# Autodesk Inventor assembly: Assembly4
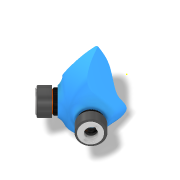
[picture p0: Inventor's stored thumbnail of the model, 180x180]
Saved by Autodesk Inventor 2021 (Build 250183000, 183)
## iProperties
Created: 2020-07-12
Part Number: Assembly4
Document SubType Name: Assembly
Designer: Derm
Author: Derm
## Documents named in this file (10)
- C:\Users\Derm\n95\v7\Assembly4.iam
- C:\Users\Derm\n95\v7\maskBodyV4Molds\thermoformedSupport.ipt
- C:\Users\Derm\n95\v7\3dpBayonetteMountV1Fastener.ipt
- C:\Users\Derm\n95\v7\3dpBayonetteMountV2.ipt
- C:\Users\Derm\n95\v7\outerMountGasket.ipt
- C:\Users\Derm\n95\v7\maskBodyV4Molds\main.ipt
- C:\Users\Derm\n95\v7\cartMount.ipt
- C:\Users\Derm\n95\v7\cartCap.ipt
- C:\Users\Derm\n95\v7\1inFilterInsert.ipt
- C:\Users\Derm\n95\v7\1inFilterInsertGasket.ipt
## Components (15 placed, 9 different names)
1. thermoformedSupport:1 — Mate:3, Mate:6, Mate:7, Mate:8, Mate:11, Mate:12, Flush:1, Flush:2
2. 3dpBayonetteMountV1Fastener:1 — Mate:5, Mate:7, Mate:10, Mate:18
3. 3dpBayonetteMountV2:1 — Mate:4, Mate:5, Mate:6, Mate:11, Mate:13, Mate:14, Mate:15
4. outerMountGasket:1 — Mate:4, Mate:10, Mate:17
5. 3dpBayonetteMountV1Fastener:2 — Mate:2, Mate:8, Mate:9, Mate:19
6. 3dpBayonetteMountV2:2 — Mate:1, Mate:3, Mate:12, Mate:16
7. outerMountGasket:2 — Mate:1, Mate:2, Mate:9
8. main:1 — Flush:1, Flush:2, Mate:14, Mate:15, Mate:16, Mate:18
9. cartMount:1 — Mate:13, Mate:17, Mate:21, Mate:22, Mate:25
10. cartMount:2 — Mate:19, Mate:20
11. cartCap:1 — Mate:21
12. cartCap:2 — Mate:20
13. 1inFilterInsert:1 — Mate:22, Flush:3, Mate:23
14. 1inFilterInsertGasket:1 — Flush:3, Mate:24, Mate:25
15. 1inFilterInsertGasket:2 — Mate:23, Mate:24
## Relationships (28: Mate 25, Flush 3)
- Mate:1: 3dpBayonetteMountV2:2 ↔ outerMountGasket:2
- Mate:2: 3dpBayonetteMountV1Fastener:2 ↔ outerMountGasket:2
- Mate:3: thermoformedSupport:1 ↔ 3dpBayonetteMountV2:2
- Mate:4: 3dpBayonetteMountV2:1 ↔ outerMountGasket:1
- Mate:5: 3dpBayonetteMountV1Fastener:1 ↔ 3dpBayonetteMountV2:1
- Mate:6: thermoformedSupport:1 ↔ 3dpBayonetteMountV2:1
- Mate:7: thermoformedSupport:1 ↔ 3dpBayonetteMountV1Fastener:1
- Mate:8: thermoformedSupport:1 ↔ 3dpBayonetteMountV1Fastener:2
- Mate:9: 3dpBayonetteMountV1Fastener:2 ↔ outerMountGasket:2
- Mate:10: 3dpBayonetteMountV1Fastener:1 ↔ outerMountGasket:1
- Mate:11: thermoformedSupport:1 ↔ 3dpBayonetteMountV2:1
- Mate:12: thermoformedSupport:1 ↔ 3dpBayonetteMountV2:2
- Flush:1: thermoformedSupport:1 ↔ main:1
- Flush:2: thermoformedSupport:1 ↔ main:1
- Mate:13: 3dpBayonetteMountV2:1 ↔ cartMount:1
- Mate:14: 3dpBayonetteMountV2:1 ↔ main:1
- Mate:15: 3dpBayonetteMountV2:1 ↔ main:1
- Mate:16: 3dpBayonetteMountV2:2 ↔ main:1
- Mate:17: outerMountGasket:1 ↔ cartMount:1
- Mate:18: 3dpBayonetteMountV1Fastener:1 ↔ main:1
- Mate:19: 3dpBayonetteMountV1Fastener:2 ↔ cartMount:2
- Mate:20: cartMount:2 ↔ cartCap:2
- Mate:21: cartMount:1 ↔ cartCap:1
- Mate:22: cartMount:1 ↔ 1inFilterInsert:1
- Flush:3: 1inFilterInsert:1 ↔ 1inFilterInsertGasket:1
- Mate:23: 1inFilterInsert:1 ↔ 1inFilterInsertGasket:2
- Mate:24: 1inFilterInsertGasket:1 ↔ 1inFilterInsertGasket:2
- Mate:25: cartMount:1 ↔ 1inFilterInsertGasket:1
